# Autodesk Inventor assembly: FRC_FieldModel_2015
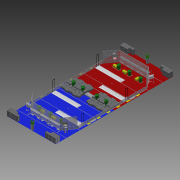
[picture p0: Inventor's stored thumbnail of the model, 180x180]
Saved by Autodesk Inventor 2015 SP1 (Build 190203100, 203)
## iProperties
Created: 2014-12-23
Part Number: FRC_FieldModel_2015
Document SubType Name: Assembly
Designer: Philip
Author: nskripsky
Title: FE-00038_ASM
Sending System: PRO/ENGINEER BY PARAMETRIC TECHNOLOGY CORPORATION, 2013230
Preprocessor: PRO/ENGINEER BY PARAMETRIC TECHNOLOGY CORPORATION, 2013230
Author: Philip
## Documents named in this file (35)
- C:\FRC 2015 Test\FRC_FieldModel_2015.iam
- C:\FRC 2015 Test\Parts\FE-00038-03.ipt
- C:\FRC 2015 Test\Parts\FE-00038-04.ipt
- C:\FRC 2015 Test\Parts\FE-00038-01_ASM.iam
- C:\FRC 2015 Test\Parts\FE-00038-02_ASM.iam
- C:\FRC 2015 Test\Parts\GE-15000_ASM.iam
- C:\FRC 2015 Test\Parts\GE-15001_ASM.iam
- C:\FRC 2015 Test\Parts\GE-15014_ASM.iam
- C:\FRC 2015 Test\Parts\FE-00038-13.ipt
- C:\FRC 2015 Test\Parts\GE-15025_ASM.iam
- C:\FRC 2015 Test\Parts\GE-15022_ASM.iam
- C:\FRC 2015 Test\Parts\GE-15023_ASM.iam
- C:\FRC 2015 Test\Parts\GE-15021_ASM.iam
- C:\FRC 2015 Test\Parts\FE-00038-05.ipt
- C:\FRC 2015 Test\Parts\FE-00038-08.ipt
- C:\FRC 2015 Test\Parts\FE-00038-09.ipt
- C:\FRC 2015 Test\Parts\FE-00038-06.ipt
- C:\FRC 2015 Test\Parts\FE-00038-07.ipt
- C:\FRC 2015 Test\Parts\FE-00038-10.ipt
- C:\FRC 2015 Test\Parts\GE-15017.ipt
- C:\FRC 2015 Test\Parts\GE-15018.ipt
- C:\FRC 2015 Test\Parts\FE-00038-11.ipt
- C:\FRC 2015 Test\Parts\FE-00038-12.ipt
- C:\FRC 2015 Test\Parts\STEP_GP_ASM.iam
- C:\FRC 2015 Test\Parts\LANDFILL_GP_ASM.iam
- C:\FRC 2015 Test\Parts\LANDFILL_GP2_ASM.iam
- C:\FRC 2015 Test\Parts\LANDFILL_GP3_ASM.iam
- C:\FRC 2015 Test\Parts\GE-15040.ipt
- C:\FRC 2015 Test\Parts\ALLIANCE_STATION_GP1_ASM.iam
- C:\FRC 2015 Test\Parts\ALLIANCE_STATION_GP2_ASM.iam
- C:\FRC 2015 Test\Parts\ALLIANCE_STATION_GP3_ASM.iam
- C:\FRC 2015 Test\Parts\YELLOW_TOTEASM_ASM.iam
- C:\FRC 2015 Test\Parts\RECYCLING_BIN_ASM.iam
- C:\FRC 2015 Test\Parts\GE-15001_ASM_Red.iam
- C:\FRC 2015 Test\Parts\GE-15000_ASM_Red.iam
## Components (93 placed, 83 different names)
1. FE-00038-03_0 — Planar:1, Planar:2, Planar:3, Planar:4, Planar:5, Planar:6, Planar:7
2. FE-00038-03_1 — Planar:8, Planar:9
3. FE-00038-04_2 — Planar:10, Planar:11
4. FE-00038-04_3 — Planar:12
5. FE-00038-01_ASM_75 [sub-assembly]
6. FE-00038-01_ASM_76 [sub-assembly]
7. FE-00038-02_ASM_155 [sub-assembly]
8. FE-00038-02_ASM_156 [sub-assembly]
9. GE-15000_ASM_190 [sub-assembly]
10. GE-15001_ASM_208 [sub-assembly]
11. GE-15000_ASM_209 [sub-assembly]
12. GE-15001_ASM_210 [sub-assembly]
13. GE-15014_ASM_220 [sub-assembly]
14. GE-15014_ASM_221 [sub-assembly]
15. GE-15014_ASM_222 [sub-assembly]
16. GE-15014_ASM_223 [sub-assembly]
17. GE-15014_ASM_224 [sub-assembly]
18. GE-15014_ASM_225 [sub-assembly]
19. GE-15014_ASM_226 [sub-assembly]
20. FE-00038-13_227
21. FE-00038-13_228
22. GE-15025_ASM_256 [sub-assembly]
23. GE-15025_ASM_257 [sub-assembly]
24. GE-15025_ASM_258 [sub-assembly]
25. GE-15025_ASM_259 [sub-assembly]
26. GE-15022_ASM_263 [sub-assembly]
27. GE-15022_ASM_264 [sub-assembly]
28. GE-15022_ASM_265 [sub-assembly]
29. GE-15022_ASM_266 [sub-assembly]
30. GE-15023_ASM_282 [sub-assembly]
31. GE-15023_ASM_283 [sub-assembly]
32. GE-15023_ASM_284 [sub-assembly]
33. GE-15023_ASM_285 [sub-assembly]
34. GE-15021_ASM_289 [sub-assembly]
35. GE-15021_ASM_290 [sub-assembly]
36. GE-15021_ASM_291 [sub-assembly]
37. GE-15021_ASM_292 [sub-assembly]
38. FE-00038-05_293
39. FE-00038-05_294
40. FE-00038-08_295
41. FE-00038-08_296
42. FE-00038-08_297
43. FE-00038-09_298
44. FE-00038-09_299
45. FE-00038-09_300
46. FE-00038-06_301
47. FE-00038-06_302
48. FE-00038-07_303
49. FE-00038-07_304
50. FE-00038-10_305
51. FE-00038-10_306
52. GE-15017_307
53. GE-15017_308
54. GE-15018_309
55. GE-15018_310
56. FE-00038-11_311
57. FE-00038-11_312
58. FE-00038-11_313
59. FE-00038-11_314
60. FE-00038-12_315
61. FE-00038-12_316
62. FE-00038-12_317
63. FE-00038-12_318
64. STEP_GP_ASM_342 [sub-assembly]
65. STEP_GP_ASM_343 [sub-assembly]
66. LANDFILL_GP_ASM_349 [sub-assembly]
67. LANDFILL_GP_ASM_350 [sub-assembly]
68. LANDFILL_GP_ASM_351 [sub-assembly]
69. LANDFILL_GP_ASM_352 [sub-assembly]
70. LANDFILL_GP2_ASM_362 [sub-assembly]
71. LANDFILL_GP2_ASM_363 [sub-assembly]
72. LANDFILL_GP3_ASM_373 [sub-assembly]
73. LANDFILL_GP3_ASM_374 [sub-assembly]
74. GE-15040_375
75. GE-15040_376
76. ALLIANCE_STATION_GP1_ASM_392 [sub-assembly]
77. ALLIANCE_STATION_GP1_ASM_393 [sub-assembly]
78. ALLIANCE_STATION_GP2_ASM_409 [sub-assembly]
79. ALLIANCE_STATION_GP2_ASM_410 [sub-assembly]
80. ALLIANCE_STATION_GP3_ASM_421 [sub-assembly]
81. ALLIANCE_STATION_GP3_ASM_422 [sub-assembly]
82. YELLOW_TOTEASM_ASM:1 [sub-assembly] — Planar:2
83. YELLOW_TOTEASM_ASM:2 [sub-assembly] — Planar:3
84. YELLOW_TOTEASM_ASM:3 [sub-assembly] — Planar:4
85. YELLOW_TOTEASM_ASM:4 [sub-assembly] — Planar:5
86. YELLOW_TOTEASM_ASM:5 [sub-assembly] — Planar:6
87. YELLOW_TOTEASM_ASM:6 [sub-assembly] — Planar:7
88. RECYCLING_BIN_ASM:1 [sub-assembly] — Planar:1
89. RECYCLING_BIN_ASM:2 [sub-assembly] — Planar:8
90. RECYCLING_BIN_ASM:3 [sub-assembly] — Planar:9
91. RECYCLING_BIN_ASM:4 [sub-assembly] — Planar:10
92. RECYCLING_BIN_ASM:5 [sub-assembly] — Planar:11
93. RECYCLING_BIN_ASM:6 [sub-assembly] — Planar:12
## Relationships (12: PlanarJoint 12)
- Planar:1: FE-00038-03_0 ↔ RECYCLING_BIN_ASM:1
- Planar:2: FE-00038-03_0 ↔ YELLOW_TOTEASM_ASM:1
- Planar:3: FE-00038-03_0 ↔ YELLOW_TOTEASM_ASM:2
- Planar:4: FE-00038-03_0 ↔ YELLOW_TOTEASM_ASM:3
- Planar:5: FE-00038-03_0 ↔ YELLOW_TOTEASM_ASM:4
- Planar:6: FE-00038-03_0 ↔ YELLOW_TOTEASM_ASM:5
- Planar:7: FE-00038-03_0 ↔ YELLOW_TOTEASM_ASM:6
- Planar:8: FE-00038-03_1 ↔ RECYCLING_BIN_ASM:2
- Planar:9: FE-00038-03_1 ↔ RECYCLING_BIN_ASM:3
- Planar:10: FE-00038-04_2 ↔ RECYCLING_BIN_ASM:4
- Planar:11: FE-00038-04_2 ↔ RECYCLING_BIN_ASM:5
- Planar:12: FE-00038-04_3 ↔ RECYCLING_BIN_ASM:6
